# Autodesk Inventor assembly: Boxv3lasercut
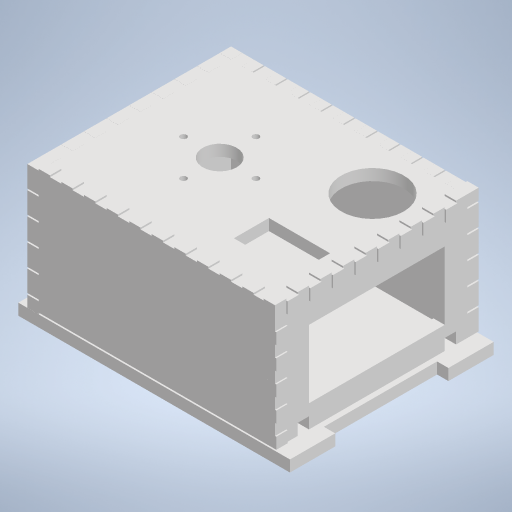
[picture p0: Inventor's stored thumbnail of the model, 512x512]
Saved by Autodesk Inventor 2024 (Build 280153000, 153)
## iProperties
Created: 2024-04-16
Part Number: Boxv3lasercut
Document SubType Name: Assembly
Designer: srika
Author: srika
## Documents named in this file (6)
- C:\Users\srika\Documents\Autodesk\Boxv2laserBottomEdge\Boxv3lasercut.iam
- C:\Users\srika\Documents\Autodesk\Boxv2laserBottomEdge\topside.ipt
- C:\Users\srika\Documents\Autodesk\Boxv2laserBottomEdge\frontbackside.ipt
- C:\Users\srika\Documents\Autodesk\Boxv2laserBottomEdge\leftrightsidehole.ipt
- C:\Users\srika\Documents\Autodesk\Boxv2laserBottomEdge\leftrightside.ipt
- C:\Users\srika\Documents\Autodesk\Boxv2laserBottomEdge\bottomside.ipt
## Components (6 placed, 5 different names)
1. topside:1 — Mate:1, Mate:2, Mate:4
2. frontbackside:1 — Mate:1
3. frontbackside:2 — Mate:2, Mate:3, Mate:5
4. leftrightsidehole:1 — Mate:3
5. leftrightside:1 — Mate:4
6. bottomside:1 — Mate:5
## Relationships (5: Mate 5)
- Mate:1: topside:1 ↔ frontbackside:1
- Mate:2: topside:1 ↔ frontbackside:2
- Mate:3: frontbackside:2 ↔ leftrightsidehole:1
- Mate:4: topside:1 ↔ leftrightside:1
- Mate:5: frontbackside:2 ↔ bottomside:1
